# Autodesk Inventor assembly: ASY PNS 750 filter-distribution-system 1200
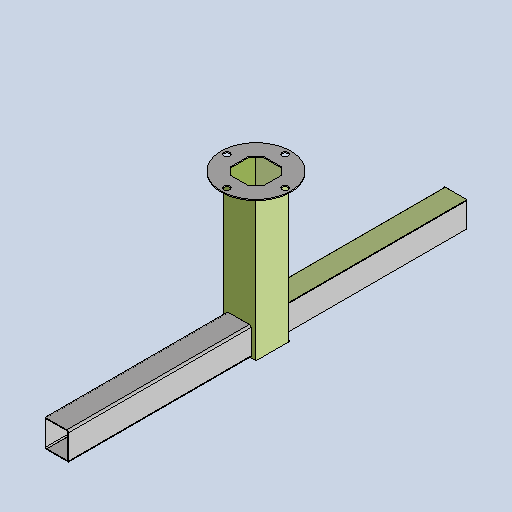
[picture p0: Inventor's stored thumbnail of the model, 512x512]
Saved by Autodesk Inventor 2025 (Build 290162010, 162A)
## iProperties
Created: 2025-06-24
Part Number: ASY PNS 750 filter-distribution-system 1200
Document SubType Name: Assembly
Designer: user
Author: user
## Documents named in this file (5)
- C:\Users\admin\YandexDisk-badmisterfox\home pc\Inventor\PNS-RESTORE\Filter D1200\ASY PNS 750 filter-distribution-system 1200.iam
- C:\Users\admin\YandexDisk-badmisterfox\home pc\Inventor\PNS-RESTORE\Filter D1200\PNS 751 DIM filter-distribution-system 1200.ipt
- C:\Users\admin\YandexDisk-badmisterfox\home pc\Inventor\PNS-RESTORE\Filter D1200\PNS 754 FDS 1200 FLANGE.ipt
- C:\Users\admin\YandexDisk-badmisterfox\home pc\Inventor\PNS-RESTORE\Filter D1200\PNS 752 FDS 1200 FLANGE 2.ipt
- C:\Users\admin\YandexDisk-badmisterfox\home pc\Inventor\PNS-RESTORE\Filter D1200\PNS 753 FDS 1200 FLANGE 3.ipt
## Components (8 placed, 4 different names)
1. Dimensions:1 — Mate:4, Mate:5
2. PNS FDS 1200 FLANGE:1 — Mate:1, Flush:1, Flush:2
3. PNS FDS 1200 FLANGE 2:1 — Rigid:1, Flush:1, Mate:2, Flush:3, Flush:4
4. PNS FDS 1200 FLANGE 2:2 — Rigid:1, Mate:1, Flush:2, Mate:3, Flush:5, Flush:6
5. PNS FDS 1200 FLANGE 3:1 — Rigid:2, Mate:2, Flush:3, Flush:4
6. PNS FDS 1200 FLANGE 3:2 — Rigid:2
7. PNS FDS 1200 FLANGE 3:3 — Mate:3, Flush:5
8. PNS FDS 1200 FLANGE 3:4 — Flush:6
## Relationships (14: Flush 6, Mate 5, WeldJoint 3)
- Rigid:1 [WeldJoint]: PNS FDS 1200 FLANGE 2:1 ↔ PNS FDS 1200 FLANGE 2:2
- Mate:1: PNS FDS 1200 FLANGE:1 ↔ PNS FDS 1200 FLANGE 2:2
- Flush:1: PNS FDS 1200 FLANGE:1 ↔ PNS FDS 1200 FLANGE 2:1
- Flush:2: PNS FDS 1200 FLANGE:1 ↔ PNS FDS 1200 FLANGE 2:2
- Rigid:2 [WeldJoint]: PNS FDS 1200 FLANGE 3:1 ↔ PNS FDS 1200 FLANGE 3:2
- Mate:2: PNS FDS 1200 FLANGE 2:1 ↔ PNS FDS 1200 FLANGE 3:1
- Flush:3: PNS FDS 1200 FLANGE 2:1 ↔ PNS FDS 1200 FLANGE 3:1
- Flush:4: PNS FDS 1200 FLANGE 2:1 ↔ PNS FDS 1200 FLANGE 3:1
- [WeldJoint]: PNS FDS 1200 FLANGE 3:3 ↔ PNS FDS 1200 FLANGE 3:4
- Mate:3: PNS FDS 1200 FLANGE 2:2 ↔ PNS FDS 1200 FLANGE 3:3
- Flush:5: PNS FDS 1200 FLANGE 2:2 ↔ PNS FDS 1200 FLANGE 3:3
- Flush:6: PNS FDS 1200 FLANGE 2:2 ↔ PNS FDS 1200 FLANGE 3:4
- Mate:4: Dimensions:1
- Mate:5: Dimensions:1
## Named parameters: d18_d14 = 0 mm
